# Autodesk Inventor assembly: Assembly2
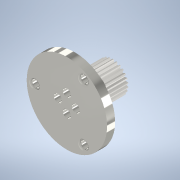
[picture p0: Inventor's stored thumbnail of the model, 180x180]
Saved by Autodesk Inventor 2022.3 (Build 263350000, 350)
## iProperties
Created: 2022-05-21
Part Number: Assembly2
Document SubType Name: Assembly
Designer: Mlees
Author: Mlees
## Documents named in this file (3)
- D:\504Engineering\Project_0000\Designs\Design_4\Created_Parts\Assembly2.iam
- D:\504Engineering\Project_0000\Designs\Design_4\Created_Parts\Planet_Gear_Output.ipt
- D:\504Engineering\Project_0000\Designs\Design_4\Created_Parts\Sun_Gear.ipt
## Components (2 placed, 2 different names)
1. Planet_Gear_Output:1 — Mate:1, Mate:2
2. Spur Gear1:1 — Mate:1, Mate:2
## Relationships (2: Mate 2)
- Mate:1: Planet_Gear_Output:1 ↔ Spur Gear1:1
- Mate:2: Planet_Gear_Output:1 ↔ Spur Gear1:1
